# Autodesk Inventor assembly: 1535_bottom_assembly
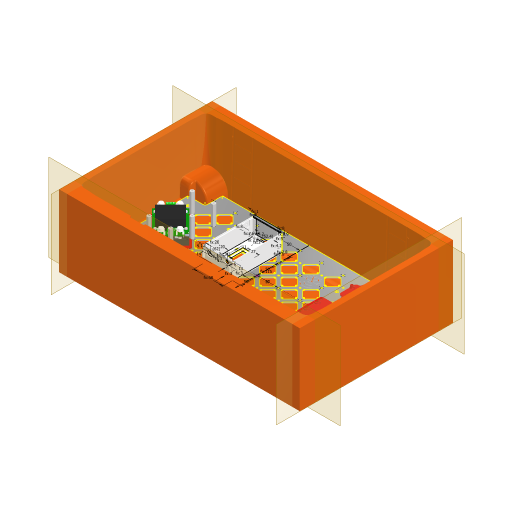
[picture p0: Inventor's stored thumbnail of the model, 512x512]
Saved by Autodesk Inventor 2023 (Build 270158000, 158)
## iProperties
Created: 2024-05-05
Part Number: 1535_bottom_assembly
Document SubType Name: Assembly
Designer: Thomas
Author: Thomas
## iProperties of the stored document tep200wircmf_3d_drawing.ipt
Created: 2022-05-11
Part Number: TEP 200  CMF
Material: Generic
Description: STEP AP214
Document SubType Name: Modeling
Designer: Thomas
Density: 1 g/cm^3
Appearance: Default
Sending System: SolidWorks 2016
Preprocessor: SwSTEP 2.0
Title: TEP 200  CMF.STEP
Revision Number: ANY
## iProperties of the stored document 98952A449_Aluminum Male-Female Threaded Hex Standoff.ipt
Company: Managed by Terraform
Created: 2021-07-10
Part Number: 98952A449_Aluminum Male-Female Threaded Hex Standoff
Material: Generic
Description: STEP AP203
Document SubType Name: Modeling
Designer: Thomas
Density: 1 g/cm^3
Appearance: Default
Sending System: SolidWorks 2017
Preprocessor: SwSTEP 2.0
Title: 98952A449_Aluminum Male-Female Threaded Hex Standoff.STEP
Author: Administrator
Revision Number: ANY
## iProperties of the stored document 1535 Bottom Tub.ipt
Created: 2019-02-13
Part Number: 1535 Bottom Tub
Material: Generic
Description: STEP AP214
Document SubType Name: Modeling
Designer: Thomas
Density: 1 g/cm^3
Appearance: Default
Sending System: SolidWorks 2016
Preprocessor: SwSTEP 2.0
Title: 1535 Bottom Tub.STEP
Revision Number: ANY
## Documents named in this file (13)
- Z:\penguin_1535_radar_case\1535_bottom_assembly.iam
- **Z:\penguin_1535_radar_case\1535_bottom_assembly.iam*LocalDocs*xAaaaqtaaAaaaaaaaAaaaqomy5d*1535 Bottom Tub.ipt
- Z:\penguin_1535_radar_case\radar_base_plate.ipt
- **Z:\penguin_1535_radar_case\1535_bottom_assembly.iam*LocalDocs*xAaaaq3daAaaaaaaaAaaaa4mzUd*98952A449_Aluminum Male-Female Threaded Hex Standoff.ipt
- Z:\penguin_1535_radar_case\amplifier_tray.ipt
- Z:\payload_enclosure_pi5\pi_shell.ipt
- Z:\penguin_1535_radar_case\traco_pa_power_mount.ipt
- **Z:\penguin_1535_radar_case\1535_bottom_assembly.iam*LocalDocs*xAaaaqjbaAaaaaaaaAaaaaqegPg*tep200wircmf_3d_drawing.ipt
- Z:\penguin_1535_radar_case\5v_power_mount.ipt
- Z:\penguin_1535_radar_case\power_distribution_mount.ipt
- Z:\penguin_1535_radar_case\reference_cad\tep200wircmf_3d_drawing.stp
- Z:\penguin_1535_radar_case\reference_cad\1535_step\1535 Bottom Tub.STEP
- Z:\penguin_1535_radar_case\reference_cad\98952A449_Aluminum Male-Female Threaded Hex Standoff.STEP
## Components (13 placed, 9 different names)
1. 1535 Bottom Tub:1 — Mate:1, Mate:2, Mate:3, Mate:4, Mate:5
2. radar_base_plate:1 — Mate:1, Mate:6, Mate:7, Insert:1, Insert:2, Insert:4, Insert:5, Insert:6, Mate:8, Insert:9, Insert:10, Insert:13, Insert:14
3. 98952A449_Aluminum Male-Female Threaded Hex Standoff:1 — Insert:1
4. 98952A449_Aluminum Male-Female Threaded Hex Standoff:2 — Insert:2, Insert:7
5. 98952A449_Aluminum Male-Female Threaded Hex Standoff:4 — Insert:4
6. 98952A449_Aluminum Male-Female Threaded Hex Standoff:5 — Insert:5, Insert:8
7. 98952A449_Aluminum Male-Female Threaded Hex Standoff:6 — Insert:6
8. amplifier_tray:1 — Insert:7, Insert:8, Mate:9
9. pi_shell:1 — Mate:8, Mate:9
10. traco_pa_power_mount:1 — Insert:9, Insert:10, Insert:11, Insert:12
11. tep200wircmf_3d_drawing:1 — Insert:11, Insert:12
12. 5v_power_mount:1 — Insert:13
13. power_distribution_mount:1 — Insert:14
## Relationships (26: Insert 13, Mate 9, Angle 4)
- Mate:1 (12.7 mm): 1535 Bottom Tub:1 ↔ radar_base_plate:1
- Mate:2: 1535 Bottom Tub:1
- Angle:1 (0 deg)
- Mate:3: 1535 Bottom Tub:1
- Angle:2 (0 deg)
- Mate:4: 1535 Bottom Tub:1
- Angle:3 (0 deg)
- Mate:5: 1535 Bottom Tub:1
- Angle:4 (0 deg)
- Mate:6 (23.5 mm): radar_base_plate:1
- Mate:7 (21 mm): radar_base_plate:1
- Insert:1: radar_base_plate:1 ↔ 98952A449_Aluminum Male-Female Threaded Hex Standoff:1
- Insert:2: radar_base_plate:1 ↔ 98952A449_Aluminum Male-Female Threaded Hex Standoff:2
- Insert:4: radar_base_plate:1 ↔ 98952A449_Aluminum Male-Female Threaded Hex Standoff:4
- Insert:5: radar_base_plate:1 ↔ 98952A449_Aluminum Male-Female Threaded Hex Standoff:5
- Insert:6: radar_base_plate:1 ↔ 98952A449_Aluminum Male-Female Threaded Hex Standoff:6
- Insert:7: 98952A449_Aluminum Male-Female Threaded Hex Standoff:2 ↔ amplifier_tray:1
- Insert:8: 98952A449_Aluminum Male-Female Threaded Hex Standoff:5 ↔ amplifier_tray:1
- Mate:8: radar_base_plate:1 ↔ pi_shell:1
- Mate:9 (35 mm): amplifier_tray:1 ↔ pi_shell:1
- Insert:9: radar_base_plate:1 ↔ traco_pa_power_mount:1
- Insert:10: radar_base_plate:1 ↔ traco_pa_power_mount:1
- Insert:11: traco_pa_power_mount:1 ↔ tep200wircmf_3d_drawing:1
- Insert:12: traco_pa_power_mount:1 ↔ tep200wircmf_3d_drawing:1
- Insert:13: radar_base_plate:1 ↔ 5v_power_mount:1
- Insert:14: radar_base_plate:1 ↔ power_distribution_mount:1
